# Autodesk Inventor assembly: vexFrisbeeShooter10
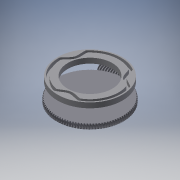
[picture p0: Inventor's stored thumbnail of the model, 180x180]
Saved by Autodesk Inventor 2016 SP1 (Build 200210100, 210)
## iProperties
Created: 2015-11-02
Part Number: vexFrisbeeShooter10
Document SubType Name: Assembly
Designer: steele
Author: steele
## Documents named in this file (3)
- C:\snobotics\CAD-Development\robSteele\FRC 2013 Ultimate Ascent\vexFrisbeeShooter10.iam
- C:\snobotics\CAD-Development\robSteele\FRC 2013 Ultimate Ascent\vexCamRing10.ipt
- C:\snobotics\CAD-Development\robSteele\FRC 2013 Ultimate Ascent\vexFrisbeeShooter10\Design Accelerator\Worm Gears1.iam
## Components (2 placed, 2 different names)
1. vexCamRing10:1 — Mate:1, Angle:1
2. Worm Gears:1 [sub-assembly] — Mate:1, Angle:1
## Relationships (2: Mate 1, Angle 1)
- Mate:1: vexCamRing10:1 ↔ Worm Gears:1
- Angle:1 (0 deg): vexCamRing10:1 ↔ Worm Gears:1
